# Autodesk Inventor assembly: X02598_LEGOmini_UpperBody
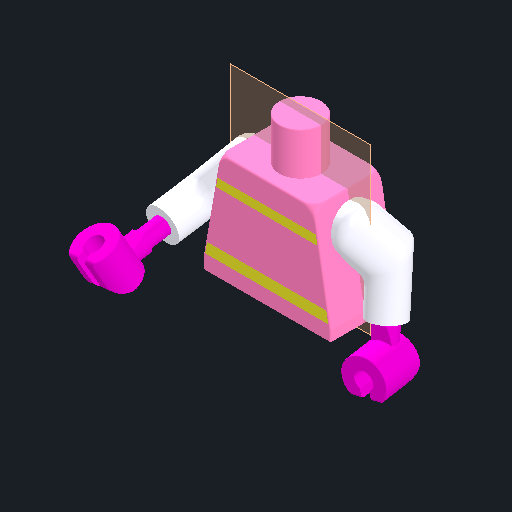
[picture p0: Inventor's stored thumbnail of the model, 512x512]
Saved by Autodesk Inventor 2022 (Build 260153000, 153)
## iProperties
Created: 2022-02-05
Part Number: X02598_LEGOmini_UpperBody
Document SubType Name: Assembly
Designer: Jason
Author: Jason
## Documents named in this file (6)
- C:\Users\User\Desktop\110033226_LEGOmini_消防隊員\110033226_LEGOmini_上半身.iam
- C:\Users\User\Desktop\110033226_LEGOmini_消防隊員\110033226_LEGOmini_上半身.ipt
- C:\Users\User\Desktop\110033226_LEGOmini_消防隊員\110033226_LEGOmini_左手臂.ipt
- C:\Users\User\Desktop\110033226_LEGOmini_消防隊員\110033226_LEGOmini_右手臂.ipt.ipt
- C:\Users\User\Desktop\110033226_LEGOmini_消防隊員\110033226_LEGOmini_手.ipt
- 110033226_LEGOmini_右手臂.ipt
## Components (5 placed, 4 different names)
1. 110033226_LEGOmini_上半身:1 — 插入:1, 插入:2
2. 110033226_LEGOmini_左手臂:1 — 插入:1, 貼合:2
3. 110033226_LEGOmini_右手臂.ipt:1 — 插入:2, 貼合:1
4. 110033226_LEGOmini_手:1 — 貼合:1
5. 110033226_LEGOmini_手:2 — 貼合:2
## Relationships (4: Insert 2, Mate 2)
- 插入:1 [Insert]: 110033226_LEGOmini_上半身:1 ↔ 110033226_LEGOmini_左手臂:1
- 插入:2 [Insert]: 110033226_LEGOmini_上半身:1 ↔ 110033226_LEGOmini_右手臂.ipt:1
- 貼合:1 [Mate]: 110033226_LEGOmini_右手臂.ipt:1 ↔ 110033226_LEGOmini_手:1
- 貼合:2 [Mate]: 110033226_LEGOmini_左手臂:1 ↔ 110033226_LEGOmini_手:2
